# Autodesk Inventor assembly: 知能ロボコン吸引部
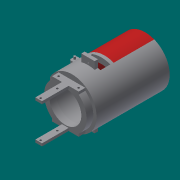
[picture p0: Inventor's stored thumbnail of the model, 180x180]
Saved by Autodesk Inventor 2013 (Build 170138000, 138)
## iProperties
Created: 2014-11-21
Part Number: 知能ロボコン吸引部
Document SubType Name: Assembly
Designer: horumo136
Author: horumo136
## Documents named in this file (5)
- C:\Users\horumo136\Documents\知能ロボコン吸引部.iam
- C:\Users\horumo136\Documents\知能ロボコン吸引部２.1.1.ipt
- C:\Users\horumo136\Documents\知能ロボコン吸引部２.1.2.ipt
- C:\Users\horumo136\Documents\3mmシャフト.ipt
- C:\Users\horumo136\Documents\知能ロボコンファン止め具.ipt
## Components (5 placed, 4 different names)
1. 知能ロボコン吸引部２.1.1:1 — メイト:1, メイト:3, メイト:4, メイト:5, メイト:6, メイト:7, メイト:8
2. 知能ロボコン吸引部２.1.2:1 — メイト:2
3. 3mmシャフト:1 — メイト:1, メイト:2
4. 知能ロボコンファン止め具:1 — メイト:3, メイト:4, メイト:5
5. 知能ロボコンファン止め具:2 — メイト:6, メイト:7, メイト:8
## Relationships (8: Mate 8)
- メイト:1 [Mate]: 知能ロボコン吸引部２.1.1:1 ↔ 3mmシャフト:1
- メイト:2 [Mate]: 知能ロボコン吸引部２.1.2:1 ↔ 3mmシャフト:1
- メイト:3 [Mate]: 知能ロボコン吸引部２.1.1:1 ↔ 知能ロボコンファン止め具:1
- メイト:4 [Mate]: 知能ロボコン吸引部２.1.1:1 ↔ 知能ロボコンファン止め具:1
- メイト:5 [Mate]: 知能ロボコン吸引部２.1.1:1 ↔ 知能ロボコンファン止め具:1
- メイト:6 [Mate]: 知能ロボコン吸引部２.1.1:1 ↔ 知能ロボコンファン止め具:2
- メイト:7 [Mate]: 知能ロボコン吸引部２.1.1:1 ↔ 知能ロボコンファン止め具:2
- メイト:8 [Mate]: 知能ロボコン吸引部２.1.1:1 ↔ 知能ロボコンファン止め具:2
